# Autodesk Inventor assembly: Lego Assembly
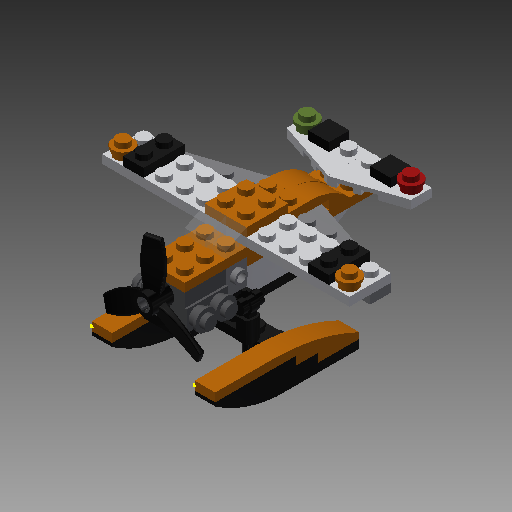
[picture p0: Inventor's stored thumbnail of the model, 512x512]
Saved by Autodesk Inventor 2017 (Build 210142000, 142)
## iProperties
Created: 2018-05-17
Part Number: Lego Assembly
Document SubType Name: Assembly
Designer: Kyle
Author: Kyle
## Documents named in this file (32)
- C:\Users\Kyle\Documents\GitHub\Lego-Project\Inventor Part Files\Lego Assembly.iam
- C:\Users\Kyle\Documents\GitHub\Lego-Project\Inventor Part Files\1x6 short black pegged.ipt
- C:\Users\Kyle\Documents\GitHub\Lego-Project\Inventor Part Files\Two Sided Piece.ipt
- C:\Users\Kyle\Documents\GitHub\Lego-Project\Inventor Part Files\2x2 tall things sticking out.ipt
- C:\Users\Kyle\Documents\GitHub\Lego-Project\Inventor Part Files\Weird circle things.ipt
- C:\Users\Kyle\Documents\GitHub\Lego-Project\Inventor Part Files\1x1 tall gray with a stick out.ipt
- C:\Users\Kyle\Documents\GitHub\Lego-Project\Inventor Part Files\1x2 tall white pegged.ipt
- C:\Users\Kyle\Documents\GitHub\Lego-Project\Inventor Part Files\1x2 short orange pegged.ipt
- C:\Users\Kyle\Documents\GitHub\Lego-Project\Inventor Part Files\3x2 most wierdest piece ever.ipt
- C:\Users\Kyle\Documents\GitHub\Lego-Project\Inventor Part Files\2x6 short orange pegged.ipt
- C:\Users\Kyle\Documents\GitHub\Lego-Project\Inventor Part Files\2x4 orange pegged.ipt
- C:\Users\Kyle\Documents\GitHub\Lego-Project\Inventor Part Files\1x1 circular almost looks like peg peg gray.ipt
- C:\Users\Kyle\Documents\GitHub\Lego-Project\Inventor Part Files\Transparent Grey Peice.ipt
- C:\Users\Kyle\Documents\GitHub\Lego-Project\Inventor Part Files\3x1 diagonal.ipt
- C:\Users\Kyle\Documents\GitHub\Lego-Project\Inventor Part Files\other diagonal piece (1).ipt
- C:\Users\Kyle\Documents\GitHub\Lego-Project\Inventor Part Files\1x1 short black smooth.ipt
- C:\Users\Kyle\Documents\GitHub\Lego-Project\Inventor Part Files\1x1 circular almost looks like peg peg green.ipt
- C:\Users\Kyle\Documents\GitHub\Lego-Project\Inventor Part Files\1x1 circular almost looks like peg peg red.ipt
- C:\Users\Kyle\Documents\GitHub\Lego-Project\Inventor Part Files\Grey triangle lego part.ipt
- C:\Users\Kyle\Documents\GitHub\Lego-Project\Inventor Part Files\opposite grey peice.ipt
- C:\Users\Kyle\Documents\GitHub\Lego-Project\Inventor Part Files\2x6 short white pegged.ipt
- C:\Users\Kyle\Documents\GitHub\Lego-Project\Inventor Part Files\2x2 short orange pegged.ipt
- C:\Users\Kyle\Documents\GitHub\Lego-Project\Inventor Part Files\2x1 curve.ipt
- C:\Users\Kyle\Documents\GitHub\Lego-Project\Inventor Part Files\Propeller.ipt
- C:\Users\Kyle\Documents\GitHub\Lego-Project\Inventor Part Files\1x2 short black pegged.ipt
- C:\Users\Kyle\Documents\GitHub\Lego-Project\Inventor Part Files\1x1 circular almost looks like peg peg orange.ipt
- C:\Users\Kyle\Documents\GitHub\Lego-Project\Inventor Part Files\hand project.ipt
- C:\Users\Kyle\Documents\GitHub\Lego-Project\Inventor Part Files\1x2 short black pegged with stick thingy.ipt
- C:\Users\Kyle\Documents\GitHub\Lego-Project\Inventor Part Files\WIERD PIECE.ipt
- C:\Users\Kyle\Documents\GitHub\Lego-Project\Inventor Part Files\1x4 short black pegged.ipt
- C:\Users\Kyle\Documents\GitHub\Lego-Project\Inventor Part Files\3x1 curve.ipt
- C:\Users\Kyle\Documents\GitHub\Lego-Project\Inventor Part Files\1x3 short orange smooth.ipt
## Components (52 placed, 31 different names)
1. 1x6 short black pegged:1 — Mate:1, Flush:1, Flush:2, Mate:3, Mate:5, Flush:4, Mate:17
2. 1x6 short black pegged:2 — Mate:1, Flush:1, Flush:2, Mate:2, Flush:3, Mate:4, Mate:8, Flush:6, Flush:9, Mate:14, Flush:10, Flush:15
3. Two Sided Piece:1 — Mate:2, Flush:3, Mate:4, Mate:6, Flush:5, Mate:9, Mate:21, Mate:22, Mate:23, Mate:24
4. Two Sided Piece:2 — Mate:3, Mate:5, Flush:4, Mate:7, Mate:25, Mate:26, Mate:27, Mate:28
5. 2x2 tall things sticking out:1 — Mate:6, Flush:5, Mate:7, Mate:11, Mate:20, Flush:18, Flush:19, Flush:20, Mate:50, Insert:2
6. Weird circle things:1 — Mate:8, Flush:6, Mate:9, Mate:12, Flush:23, Insert:5, Insert:6
7. 1x1 tall gray with a stick out:1 — Mate:10, Flush:7, Flush:8, Flush:9, Mate:11, Mate:12, Mate:13, Mate:15, Flush:11
8. 1x1 tall gray with a stick out:2 — Mate:10, Flush:7, Flush:8
9. 1x2 tall white pegged:1 — Mate:13, Mate:14, Flush:10, Flush:12, Mate:18
10. 1x2 short orange pegged:1 — Mate:15, Flush:11, Flush:12, Mate:19, Flush:16
11. 1x2 tall white pegged:2 — Mate:16, Flush:13, Flush:14, Mate:17, Flush:15, Mate:18, Flush:17
12. 3x2 most wierdest piece ever:1 — Mate:16, Flush:13, Flush:14
13. 2x6 short orange pegged:1 — Mate:19, Flush:16, Flush:17, Flush:26, Mate:32, Flush:27, Mate:39, Mate:48, Flush:43
14. 2x4 orange pegged:1 — Mate:20, Flush:18, Flush:19, Flush:22, Mate:30, Mate:38, Flush:35, Flush:39
15. 1x1 circular almost looks like peg peg gray:1 — Mate:26, Mate:27
16. 1x1 circular almost looks like peg peg gray:2 — Mate:25, Mate:28
17. 1x1 circular almost looks like peg peg gray:3 — Mate:21, Mate:22
18. 1x1 circular almost looks like peg peg gray:4 — Mate:23, Mate:24
19. Transparent Grey Peice:1 — Mate:29, Flush:21, Flush:23
20. Transparent Grey Peice:2 — Mate:29, Flush:20, Flush:21, Flush:22, Mate:30, Mate:42, Mate:43
21. 3x1 diagonal:1 — Mate:31, Flush:24, Flush:25, Flush:26, Flush:27, Flush:30, Flush:31, Mate:35, Insert:1, Mate:49
22. other diagonal piece (1):1 — Mate:31, Flush:24, Flush:25, Mate:32, Mate:34, Mate:36
23. 1x1 short black smooth:1 — Mate:33, Flush:28, Flush:29
24. 1x1 short black smooth:2 — Mate:33, Flush:28, Flush:29, Flush:30, Mate:34, Flush:31
25. 1x1 circular almost looks like peg peg green:1 — Flush:32, Mate:36
26. 1x1 circular almost looks like peg peg red:1 — Flush:32, Mate:35, Insert:1
27. Grey triangle lego part:1 — Mate:37, Flush:33, Flush:34, Mate:38, Mate:39, Mate:41
28. opposite grey peice:1 — Mate:37, Flush:33, Flush:34, Flush:35, Flush:38, Mate:46
29. 2x6 short white pegged:1 — Mate:40, Flush:36, Flush:37, Mate:44, Flush:48, Mate:51, Insert:3
30. 2x6 short white pegged:2 — Mate:40, Flush:36, Flush:37, Mate:41, Mate:42, Flush:38, Flush:46, Flush:47, Insert:4
31. 2x2 short orange pegged:1 — Mate:43, Flush:39, Mate:44, Mate:45, Flush:40
32. 1x2 short orange pegged:2 — Mate:45, Mate:46, Flush:40
33. 2x1 curve:1 — Mate:47, Flush:41, Flush:42
34. 2x1 curve:2 — Mate:47, Flush:41, Flush:42, Mate:48, Flush:43, Mate:49
35. Propeller:1 — Mate:50, Insert:2
36. 1x2 short black pegged:1 — Flush:44, Flush:45, Flush:48, Mate:51
37. 1x2 short black pegged:2 — Flush:44, Flush:45, Flush:46, Flush:47
38. 1x1 circular almost looks like peg peg orange:1 — Flush:49, Insert:3
39. 1x1 circular almost looks like peg peg orange:2 — Flush:49, Insert:4
40. hand project:1 — Flush:50, Flush:51, Insert:6, Insert:8
41. hand project:2 — Flush:50, Flush:51, Insert:5, Insert:7, Insert:9
42. 1x2 short black pegged with stick thingy:1 — Flush:52, Flush:53, Insert:8, Flush:58, Flush:62
43. 1x2 short black pegged with stick thingy:2 — Flush:52, Flush:53, Insert:7, Flush:56, Flush:57, Mate:52, Mate:58, Insert:9
44. WIERD PIECE:1 — Flush:54, Flush:55, Flush:58, Mate:53, Flush:67, Flush:72
45. WIERD PIECE:2 — Flush:54, Flush:55, Flush:56, Flush:57, Mate:52, Flush:61, Mate:54, Flush:63, Mate:56, Flush:66, Flush:71, Flush:73
46. 1x4 short black pegged:1 — Flush:59, Flush:60, Flush:62, Mate:53
47. 1x4 short black pegged:2 — Flush:59, Flush:60, Flush:61, Mate:54, Mate:55, Flush:68, Mate:57
48. 1x6 short black pegged:3 — Flush:63, Mate:55, Mate:56
49. 3x1 curve:1 — Flush:64, Flush:65, Flush:67
50. 3x1 curve:2 — Flush:64, Flush:65, Flush:66, Flush:68, Mate:57
51. 1x3 short orange smooth:1 — Flush:69, Flush:70, Flush:72
52. 1x3 short orange smooth:2 — Flush:69, Flush:70, Flush:71, Flush:73, Mate:58
## Relationships (140: Flush 73, Mate 58, Insert 9)
- Mate:1: 1x6 short black pegged:1 ↔ 1x6 short black pegged:2
- Flush:1: 1x6 short black pegged:1 ↔ 1x6 short black pegged:2
- Flush:2: 1x6 short black pegged:1 ↔ 1x6 short black pegged:2
- Mate:2: 1x6 short black pegged:2 ↔ Two Sided Piece:1
- Mate:3: 1x6 short black pegged:1 ↔ Two Sided Piece:2
- Flush:3: 1x6 short black pegged:2 ↔ Two Sided Piece:1
- Mate:4: 1x6 short black pegged:2 ↔ Two Sided Piece:1
- Mate:5: 1x6 short black pegged:1 ↔ Two Sided Piece:2
- Flush:4: 1x6 short black pegged:1 ↔ Two Sided Piece:2
- Mate:6: Two Sided Piece:1 ↔ 2x2 tall things sticking out:1
- Flush:5: Two Sided Piece:1 ↔ 2x2 tall things sticking out:1
- Mate:7: Two Sided Piece:2 ↔ 2x2 tall things sticking out:1
- Mate:8: 1x6 short black pegged:2 ↔ Weird circle things:1
- Flush:6: 1x6 short black pegged:2 ↔ Weird circle things:1
- Mate:9: Two Sided Piece:1 ↔ Weird circle things:1
- Mate:10: 1x1 tall gray with a stick out:1 ↔ 1x1 tall gray with a stick out:2
- Flush:7: 1x1 tall gray with a stick out:1 ↔ 1x1 tall gray with a stick out:2
- Flush:8: 1x1 tall gray with a stick out:1 ↔ 1x1 tall gray with a stick out:2
- Flush:9: 1x6 short black pegged:2 ↔ 1x1 tall gray with a stick out:1
- Mate:11: 2x2 tall things sticking out:1 ↔ 1x1 tall gray with a stick out:1
- Mate:12: Weird circle things:1 ↔ 1x1 tall gray with a stick out:1
- Mate:13: 1x1 tall gray with a stick out:1 ↔ 1x2 tall white pegged:1
- Mate:14: 1x6 short black pegged:2 ↔ 1x2 tall white pegged:1
- Flush:10: 1x6 short black pegged:2 ↔ 1x2 tall white pegged:1
- Mate:15: 1x1 tall gray with a stick out:1 ↔ 1x2 short orange pegged:1
- Flush:11: 1x1 tall gray with a stick out:1 ↔ 1x2 short orange pegged:1
- Flush:12: 1x2 tall white pegged:1 ↔ 1x2 short orange pegged:1
- Mate:16: 1x2 tall white pegged:2 ↔ 3x2 most wierdest piece ever:1
- Flush:13: 1x2 tall white pegged:2 ↔ 3x2 most wierdest piece ever:1
- Flush:14: 1x2 tall white pegged:2 ↔ 3x2 most wierdest piece ever:1
- Mate:17: 1x6 short black pegged:1 ↔ 1x2 tall white pegged:2
- Flush:15: 1x6 short black pegged:2 ↔ 1x2 tall white pegged:2
- Mate:18: 1x2 tall white pegged:1 ↔ 1x2 tall white pegged:2
- Mate:19: 1x2 short orange pegged:1 ↔ 2x6 short orange pegged:1
- Flush:16: 1x2 short orange pegged:1 ↔ 2x6 short orange pegged:1
- Flush:17: 1x2 tall white pegged:2 ↔ 2x6 short orange pegged:1
- Mate:20: 2x2 tall things sticking out:1 ↔ 2x4 orange pegged:1
- Flush:18: 2x2 tall things sticking out:1 ↔ 2x4 orange pegged:1
- Flush:19: 2x2 tall things sticking out:1 ↔ 2x4 orange pegged:1
- Mate:21: Two Sided Piece:1 ↔ 1x1 circular almost looks like peg peg gray:3
- Mate:22: Two Sided Piece:1 ↔ 1x1 circular almost looks like peg peg gray:3
- Mate:23: Two Sided Piece:1 ↔ 1x1 circular almost looks like peg peg gray:4
- Mate:24: Two Sided Piece:1 ↔ 1x1 circular almost looks like peg peg gray:4
- Mate:25: Two Sided Piece:2 ↔ 1x1 circular almost looks like peg peg gray:2
- Mate:26: Two Sided Piece:2 ↔ 1x1 circular almost looks like peg peg gray:1
- Mate:27: Two Sided Piece:2 ↔ 1x1 circular almost looks like peg peg gray:1
- Mate:28: Two Sided Piece:2 ↔ 1x1 circular almost looks like peg peg gray:2
- Mate:29: Transparent Grey Peice:1 ↔ Transparent Grey Peice:2
- Flush:20: 2x2 tall things sticking out:1 ↔ Transparent Grey Peice:2
- Flush:21: Transparent Grey Peice:1 ↔ Transparent Grey Peice:2
- Flush:22: 2x4 orange pegged:1 ↔ Transparent Grey Peice:2
- Mate:30: 2x4 orange pegged:1 ↔ Transparent Grey Peice:2
- Flush:23: Weird circle things:1 ↔ Transparent Grey Peice:1
- Mate:31: 3x1 diagonal:1 ↔ other diagonal piece (1):1
- Flush:24: 3x1 diagonal:1 ↔ other diagonal piece (1):1
- Flush:25: 3x1 diagonal:1 ↔ other diagonal piece (1):1
- Flush:26: 2x6 short orange pegged:1 ↔ 3x1 diagonal:1
- Mate:32: 2x6 short orange pegged:1 ↔ other diagonal piece (1):1
- Flush:27 (-15.5956 mm): 2x6 short orange pegged:1 ↔ 3x1 diagonal:1
- Mate:33 (15.5956 mm): 1x1 short black smooth:1 ↔ 1x1 short black smooth:2
- Flush:28: 1x1 short black smooth:1 ↔ 1x1 short black smooth:2
- Flush:29: 1x1 short black smooth:1 ↔ 1x1 short black smooth:2
- Flush:30: 3x1 diagonal:1 ↔ 1x1 short black smooth:2
- Mate:34: other diagonal piece (1):1 ↔ 1x1 short black smooth:2
- Flush:31 (7.7978 mm): 3x1 diagonal:1 ↔ 1x1 short black smooth:2
- Flush:32: 1x1 circular almost looks like peg peg green:1 ↔ 1x1 circular almost looks like peg peg red:1
- Mate:35: 3x1 diagonal:1 ↔ 1x1 circular almost looks like peg peg red:1
- Mate:36: other diagonal piece (1):1 ↔ 1x1 circular almost looks like peg peg green:1
- Insert:1: 3x1 diagonal:1 ↔ 1x1 circular almost looks like peg peg red:1
- Mate:37: Grey triangle lego part:1 ↔ opposite grey peice:1
- Flush:33: Grey triangle lego part:1 ↔ opposite grey peice:1
- Flush:34: Grey triangle lego part:1 ↔ opposite grey peice:1
- Mate:38: 2x4 orange pegged:1 ↔ Grey triangle lego part:1
- Mate:39: 2x6 short orange pegged:1 ↔ Grey triangle lego part:1
- Flush:35 (-38.989 mm): 2x4 orange pegged:1 ↔ opposite grey peice:1
- Mate:40: 2x6 short white pegged:1 ↔ 2x6 short white pegged:2
- Flush:36: 2x6 short white pegged:1 ↔ 2x6 short white pegged:2
- Flush:37: 2x6 short white pegged:1 ↔ 2x6 short white pegged:2
- Mate:41: Grey triangle lego part:1 ↔ 2x6 short white pegged:2
- Mate:42: Transparent Grey Peice:2 ↔ 2x6 short white pegged:2
- Flush:38: opposite grey peice:1 ↔ 2x6 short white pegged:2
- Mate:43: Transparent Grey Peice:2 ↔ 2x2 short orange pegged:1
- Flush:39: 2x4 orange pegged:1 ↔ 2x2 short orange pegged:1
- Mate:44: 2x6 short white pegged:1 ↔ 2x2 short orange pegged:1
- Mate:45: 2x2 short orange pegged:1 ↔ 1x2 short orange pegged:2
- Mate:46: opposite grey peice:1 ↔ 1x2 short orange pegged:2
- Flush:40: 2x2 short orange pegged:1 ↔ 1x2 short orange pegged:2
- Mate:47: 2x1 curve:1 ↔ 2x1 curve:2
- Flush:41: 2x1 curve:1 ↔ 2x1 curve:2
- Flush:42: 2x1 curve:1 ↔ 2x1 curve:2
- Mate:48: 2x6 short orange pegged:1 ↔ 2x1 curve:2
- Flush:43: 2x6 short orange pegged:1 ↔ 2x1 curve:2
- Mate:49 (-23.3934 mm): 3x1 diagonal:1 ↔ 2x1 curve:2
- Mate:50: 2x2 tall things sticking out:1 ↔ Propeller:1
- Insert:2: 2x2 tall things sticking out:1 ↔ Propeller:1
- Flush:44: 1x2 short black pegged:1 ↔ 1x2 short black pegged:2
- Flush:45: 1x2 short black pegged:1 ↔ 1x2 short black pegged:2
- Flush:46: 2x6 short white pegged:2 ↔ 1x2 short black pegged:2
- Flush:47 (7.7978 mm): 2x6 short white pegged:2 ↔ 1x2 short black pegged:2
- Flush:48 (7.7978 mm): 2x6 short white pegged:1 ↔ 1x2 short black pegged:1
- Mate:51: 2x6 short white pegged:1 ↔ 1x2 short black pegged:1
- Flush:49: 1x1 circular almost looks like peg peg orange:1 ↔ 1x1 circular almost looks like peg peg orange:2
- Insert:3: 2x6 short white pegged:1 ↔ 1x1 circular almost looks like peg peg orange:1
- Insert:4: 2x6 short white pegged:2 ↔ 1x1 circular almost looks like peg peg orange:2
- Flush:50: hand project:1 ↔ hand project:2
- Flush:51: hand project:1 ↔ hand project:2
- Insert:5: Weird circle things:1 ↔ hand project:2
- Insert:6: Weird circle things:1 ↔ hand project:1
- Flush:52: 1x2 short black pegged with stick thingy:1 ↔ 1x2 short black pegged with stick thingy:2
- Flush:53: 1x2 short black pegged with stick thingy:1 ↔ 1x2 short black pegged with stick thingy:2
- Insert:7: hand project:2 ↔ 1x2 short black pegged with stick thingy:2
- Insert:8: hand project:1 ↔ 1x2 short black pegged with stick thingy:1
- Flush:54: WIERD PIECE:1 ↔ WIERD PIECE:2
- Flush:55: WIERD PIECE:1 ↔ WIERD PIECE:2
- Flush:56: 1x2 short black pegged with stick thingy:2 ↔ WIERD PIECE:2
- Flush:57: 1x2 short black pegged with stick thingy:2 ↔ WIERD PIECE:2
- Mate:52: 1x2 short black pegged with stick thingy:2 ↔ WIERD PIECE:2
- Flush:58: 1x2 short black pegged with stick thingy:1 ↔ WIERD PIECE:1
- Flush:59: 1x4 short black pegged:1 ↔ 1x4 short black pegged:2
- Flush:60: 1x4 short black pegged:1 ↔ 1x4 short black pegged:2
- Flush:61: WIERD PIECE:2 ↔ 1x4 short black pegged:2
- Flush:62: 1x2 short black pegged with stick thingy:1 ↔ 1x4 short black pegged:1
- Mate:53: WIERD PIECE:1 ↔ 1x4 short black pegged:1
- Mate:54: WIERD PIECE:2 ↔ 1x4 short black pegged:2
- Flush:63: WIERD PIECE:2 ↔ 1x6 short black pegged:3
- Mate:55: 1x4 short black pegged:2 ↔ 1x6 short black pegged:3
- Mate:56: WIERD PIECE:2 ↔ 1x6 short black pegged:3
- Flush:64: 3x1 curve:1 ↔ 3x1 curve:2
- Flush:65: 3x1 curve:1 ↔ 3x1 curve:2
- Flush:66: WIERD PIECE:2 ↔ 3x1 curve:2
- Flush:67: WIERD PIECE:1 ↔ 3x1 curve:1
- Flush:68: 1x4 short black pegged:2 ↔ 3x1 curve:2
- Mate:57: 1x4 short black pegged:2 ↔ 3x1 curve:2
- Flush:69: 1x3 short orange smooth:1 ↔ 1x3 short orange smooth:2
- Flush:70: 1x3 short orange smooth:1 ↔ 1x3 short orange smooth:2
- Flush:71: WIERD PIECE:2 ↔ 1x3 short orange smooth:2
- Flush:72: WIERD PIECE:1 ↔ 1x3 short orange smooth:1
- Flush:73: WIERD PIECE:2 ↔ 1x3 short orange smooth:2
- Mate:58: 1x2 short black pegged with stick thingy:2 ↔ 1x3 short orange smooth:2
- Insert:9: hand project:2 ↔ 1x2 short black pegged with stick thingy:2
